# Autodesk Inventor assembly: Body Chassis Assembly
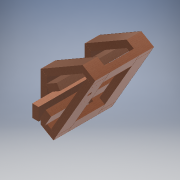
[picture p0: Inventor's stored thumbnail of the model, 180x180]
Saved by Autodesk Inventor 2017 (Build 210142000, 142)
## iProperties
Created: 2018-10-18
Part Number: Body Chassis Assembly
Document SubType Name: Assembly
Designer: Dell
Author: Dell
## Documents named in this file (7)
- C:\Users\Dell\Documents\GitHub\tr2\Body\Body Chassis Assembly.iam
- C:\Users\Dell\Documents\GitHub\tr2\Body\BO03.ipt
- C:\Users\Dell\Documents\GitHub\tr2\Body\BO14.ipt
- C:\Users\Dell\Documents\GitHub\tr2\Body\BO15.ipt
- C:\Users\Dell\Documents\GitHub\tr2\Base\BA07.ipt
- C:\Users\Dell\Documents\GitHub\tr2\Body\BO18.ipt
- C:\Users\Dell\Documents\GitHub\tr2\Body\BO19.ipt
## Components (15 placed, 6 different names)
1. BO03:2 — Mate:17, Mate:25, Flush:29, Flush:30, Flush:31, Flush:34, Flush:35, Mate:27, Mate:52
2. BO14:1 — Flush:27, Flush:28, Mate:24, Flush:31, Mate:26, Flush:32, Flush:33, Mate:50, Flush:51, Mate:51, Flush:53, Flush:58
3. BO15:1 — Mate:17, Flush:58, Mate:53
4. BO15:2 — Mate:47, Flush:55, Mate:55
5. BO15:3 — Mate:46, Flush:57, Mate:54
6. BA07:1 — Flush:27, Flush:28, Mate:24, Mate:30, Flush:39, Mate:31, Flush:52, Mate:55
7. BA07:2 — Mate:25, Flush:29, Flush:30, Mate:34, Flush:41, Mate:35, Flush:56
8. BA07:3 — Mate:26, Flush:32, Flush:33, Flush:54, Mate:53, Mate:54
9. BA07:4 — Flush:34, Flush:35, Mate:27, Mate:37
10. BO18:1 — Mate:30, Flush:39, Mate:31, Mate:32, Flush:40, Mate:33, Flush:55
11. BO18:2 — Mate:32, Flush:40, Mate:33, Flush:57
12. BO18:3 — Mate:34, Flush:41, Mate:35, Mate:36, Flush:42, Mate:47
13. BO18:4 — Mate:36, Flush:42, Mate:37, Mate:46
14. BO19:1 — Mate:50, Flush:51, Flush:52, Mate:52, Flush:56
15. BO19:2 — Mate:51, Flush:53, Flush:54
## Relationships (42: Mate 21, Flush 21)
- Mate:17: BO03:2 ↔ BO15:1
- Flush:27: BO14:1 ↔ BA07:1
- Flush:28: BO14:1 ↔ BA07:1
- Mate:24: BO14:1 ↔ BA07:1
- Mate:25: BO03:2 ↔ BA07:2
- Flush:29: BO03:2 ↔ BA07:2
- Flush:30: BO03:2 ↔ BA07:2
- Flush:31: BO03:2 ↔ BO14:1
- Mate:26: BO14:1 ↔ BA07:3
- Flush:32: BO14:1 ↔ BA07:3
- Flush:33: BO14:1 ↔ BA07:3
- Flush:34: BO03:2 ↔ BA07:4
- Flush:35: BO03:2 ↔ BA07:4
- Mate:27: BO03:2 ↔ BA07:4
- Mate:30: BA07:1 ↔ BO18:1
- Flush:39: BA07:1 ↔ BO18:1
- Mate:31: BA07:1 ↔ BO18:1
- Mate:32: BO18:1 ↔ BO18:2
- Flush:40: BO18:1 ↔ BO18:2
- Mate:33: BO18:1 ↔ BO18:2
- Mate:34: BA07:2 ↔ BO18:3
- Flush:41: BA07:2 ↔ BO18:3
- Mate:35: BA07:2 ↔ BO18:3
- Mate:36: BO18:3 ↔ BO18:4
- Flush:42: BO18:3 ↔ BO18:4
- Mate:37: BA07:4 ↔ BO18:4
- Mate:46: BO15:3 ↔ BO18:4
- Mate:47: BO15:2 ↔ BO18:3
- Mate:50: BO14:1 ↔ BO19:1
- Flush:51: BO14:1 ↔ BO19:1
- Flush:52: BA07:1 ↔ BO19:1
- Mate:51: BO14:1 ↔ BO19:2
- Flush:53: BO14:1 ↔ BO19:2
- Flush:54: BA07:3 ↔ BO19:2
- Mate:52: BO03:2 ↔ BO19:1
- Flush:55: BO15:2 ↔ BO18:1
- Flush:56: BA07:2 ↔ BO19:1
- Flush:57: BO15:3 ↔ BO18:2
- Flush:58: BO14:1 ↔ BO15:1
- Mate:53 (101.6 mm): BO15:1 ↔ BA07:3
- Mate:54 (76.2 mm): BO15:3 ↔ BA07:3
- Mate:55 (76.2 mm): BO15:2 ↔ BA07:1
